# Autodesk Inventor assembly: motorchasisholder1Ass
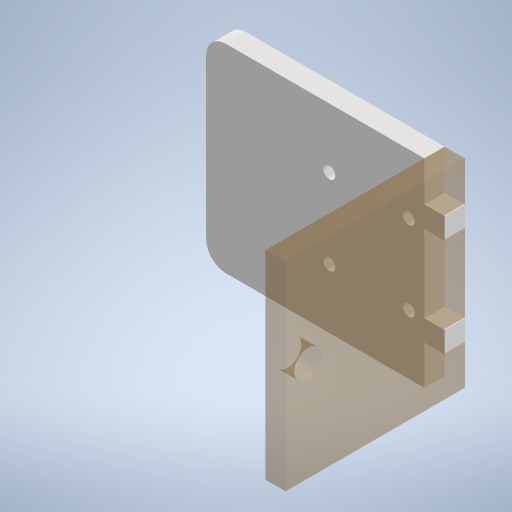
[picture p0: Inventor's stored thumbnail of the model, 512x512]
Saved by Autodesk Inventor 2023.2 (Build 272271000, 271)
## iProperties
Created: 2024-08-15
Part Number: motorchasisholder1Ass
Document SubType Name: Assembly
Designer: PC
Author: PC
## Documents named in this file (3)
- C:\Users\PC\Desktop\Kinghts mobile platform\motorchasisholder1Ass.iam
- C:\Users\PC\Desktop\Kinghts mobile platform\motorholder1A.ipt
- C:\Users\PC\Desktop\Kinghts mobile platform\motor chassis holder1.ipt
## Components (2 placed, 2 different names)
1. motorholder1A:1 — Flush:1, Flush:2, Mate:1
2. motor chassis holder1:1 — Flush:1, Flush:2, Mate:1
## Relationships (3: Flush 2, Mate 1)
- Flush:1: motorholder1A:1 ↔ motor chassis holder1:1
- Flush:2: motorholder1A:1 ↔ motor chassis holder1:1
- Mate:1: motorholder1A:1 ↔ motor chassis holder1:1
